# Autodesk Inventor assembly: MainPCB_RPI_assemblyt
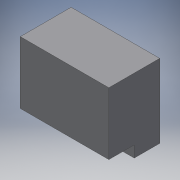
[picture p0: Inventor's stored thumbnail of the model, 180x180]
Saved by Autodesk Inventor 2019.4 (Build 234330000, 330)
## iProperties
Created: 2020-03-12
Part Number: MainPCB_RPI_assemblyt
Document SubType Name: Assembly
Designer: Jorian Bruslind
Author: Jorian Bruslind
## Documents named in this file (4)
- C:\Users\Jorian Bruslind\Documents\GitHub\ECE44x_Senior_Design\Design files\Delta Robot Arm\Inventor Files\Custom_Delta\MainPCB_RPI_assemblyt.iam
- C:\Users\Jorian Bruslind\Documents\GitHub\ECE44x_Senior_Design\Design files\Delta Robot Arm\Inventor Files\raspberry-pi-4-model-b-1.snapshot.3\Raspberry Pi 4 Model B.iam
- C:\Users\Jorian Bruslind\Documents\GitHub\ECE44x_Senior_Design\Design files\Delta Robot Arm\Inventor Files\Custom_Delta\MainPCB_RPI_Case.ipt
- C:\Users\Jorian Bruslind\Documents\GitHub\ECE44x_Senior_Design\Design files\Delta Robot Arm\PCB Files\Automated Microbial Analysis - Main Board\ExportSTEP\Main_Board.iam
## Components (3 placed, 3 different names)
1. Raspberry Pi 4 Model B:1 [sub-assembly] — Mate:1, Mate:2, Mate:3, Mate:4, Mate:5
2. MainPCB_RPI_Case:1 — Mate:1, Mate:2, Mate:3, Mate:6
3. Main_Board:1 [sub-assembly] — Mate:4, Mate:5, Mate:6
## Relationships (6: Mate 6)
- Mate:1 (4 mm): Raspberry Pi 4 Model B:1 ↔ MainPCB_RPI_Case:1
- Mate:2: Raspberry Pi 4 Model B:1 ↔ MainPCB_RPI_Case:1
- Mate:3: Raspberry Pi 4 Model B:1 ↔ MainPCB_RPI_Case:1
- Mate:4 (29 mm): Raspberry Pi 4 Model B:1 ↔ Main_Board:1
- Mate:5: Raspberry Pi 4 Model B:1 ↔ Main_Board:1
- Mate:6: MainPCB_RPI_Case:1 ↔ Main_Board:1
